# Autodesk Inventor assembly: Full Chassis with Arduino, Gyro, 1 inch Arms, and Konylak Wheels
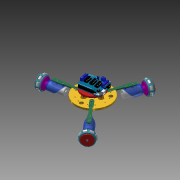
[picture p0: Inventor's stored thumbnail of the model, 180x180]
Saved by Autodesk Inventor 2014 (Build 180170000, 170)
## iProperties
Created: 2014-02-14
Part Number: Full Chassis with Arduino, Gyro, 1 inch Arms, and Konylak Wheels
Document SubType Name: Assembly
Designer: Spooner
Author: Spooner
## Documents named in this file (6)
- C:\Users\Spooner\Documents\Inventor\FerretBall Robot\3Pod\Inventor 2014 Files\Full Chassis with Arduino, Gyro, 1 inch Arms, and Konylak Wheels.iam
- C:\Users\Spooner\Documents\Inventor\FerretBall Robot\3Pod\Inventor 2014 Files\Main Body with Arduino and Gyro Mounts.iam
- C:\Users\Spooner\Documents\Inventor\Content Center Files\R2014\en-US\JIS B 1111(1)\JIS B 1111 - M3x10(1).ipt
- C:\Users\Spooner\Documents\Inventor\Content Center Files\R2014\en-US\JIS B 1181 U\JIS B 1181 - B M3.ipt
- C:\Users\Spooner\Documents\Inventor\FerretBall Robot\3Pod\Inventor 2014 Files\Full Motor Arm (1 inch) with Kornylak Wheel.iam
- C:\Users\Spooner\Documents\Inventor\FerretBall Robot\3Pod\Inventor 2014 Files\Adafruit Motor Sheild 1.2.ipt
## Components (17 placed, 5 different names)
1. Main Body with Arduino and Gyro Mounts:1 [sub-assembly] — Insert:10, Insert:11, Insert:12, Insert:13, Insert:14, Insert:15, Insert:16, Insert:17, Insert:18, Mate:4, Angle:7, Mate:5
2. JIS B 1111 M3x10:1 — Insert:11, Mate:3
3. JIS B 1111 M3x10:2 — Insert:10
4. JIS B 1111 M3x10:3 — Insert:15, Mate:1
5. JIS B 1111 M3x10:4 — Insert:14
6. JIS B 1111 M3x10:5 — Insert:13, Mate:2
7. JIS B 1111 M3x10:6 — Insert:12
8. JIS B 1181 (unchamfered) - Metric B M3:1 — Insert:21, Angle:1
9. JIS B 1181 (unchamfered) - Metric B M3:2 — Insert:24, Angle:6
10. JIS B 1181 (unchamfered) - Metric B M3:3 — Insert:19, Angle:2
11. JIS B 1181 (unchamfered) - Metric B M3:4 — Insert:20, Angle:3
12. JIS B 1181 (unchamfered) - Metric B M3:5 — Insert:22, Angle:4
13. JIS B 1181 (unchamfered) - Metric B M3:6 — Insert:23, Angle:5
14. Full Motor Arm (1 inch) with Kornylak Wheel:1 [sub-assembly] — Insert:18, Mate:3, Insert:21, Angle:1, Insert:24, Angle:6
15. Full Motor Arm (1 inch) with Kornylak Wheel:2 [sub-assembly] — Insert:17, Mate:2, Insert:22, Insert:23, Angle:4, Angle:5
16. Full Motor Arm (1 inch) with Kornylak Wheel:3 [sub-assembly] — Insert:16, Mate:1, Insert:19, Insert:20, Angle:2, Angle:3
17. Adafruit Motor Sheild 1.2:1 — Mate:4, Angle:7, Mate:5
## Relationships (27: Insert 15, Angle 7, Mate 5)
- Insert:10: Main Body with Arduino and Gyro Mounts:1 ↔ JIS B 1111 M3x10:2
- Insert:11: Main Body with Arduino and Gyro Mounts:1 ↔ JIS B 1111 M3x10:1
- Insert:12: Main Body with Arduino and Gyro Mounts:1 ↔ JIS B 1111 M3x10:6
- Insert:13: Main Body with Arduino and Gyro Mounts:1 ↔ JIS B 1111 M3x10:5
- Insert:14: Main Body with Arduino and Gyro Mounts:1 ↔ JIS B 1111 M3x10:4
- Insert:15: Main Body with Arduino and Gyro Mounts:1 ↔ JIS B 1111 M3x10:3
- Insert:16: Main Body with Arduino and Gyro Mounts:1 ↔ Full Motor Arm (1 inch) with Kornylak Wheel:3
- Mate:1: JIS B 1111 M3x10:3 ↔ Full Motor Arm (1 inch) with Kornylak Wheel:3
- Insert:17: Main Body with Arduino and Gyro Mounts:1 ↔ Full Motor Arm (1 inch) with Kornylak Wheel:2
- Mate:2: JIS B 1111 M3x10:5 ↔ Full Motor Arm (1 inch) with Kornylak Wheel:2
- Insert:18: Main Body with Arduino and Gyro Mounts:1 ↔ Full Motor Arm (1 inch) with Kornylak Wheel:1
- Mate:3: JIS B 1111 M3x10:1 ↔ Full Motor Arm (1 inch) with Kornylak Wheel:1
- Insert:19: JIS B 1181 (unchamfered) - Metric B M3:3 ↔ Full Motor Arm (1 inch) with Kornylak Wheel:3
- Insert:20: JIS B 1181 (unchamfered) - Metric B M3:4 ↔ Full Motor Arm (1 inch) with Kornylak Wheel:3
- Insert:21: JIS B 1181 (unchamfered) - Metric B M3:1 ↔ Full Motor Arm (1 inch) with Kornylak Wheel:1
- Insert:22: JIS B 1181 (unchamfered) - Metric B M3:5 ↔ Full Motor Arm (1 inch) with Kornylak Wheel:2
- Insert:23: JIS B 1181 (unchamfered) - Metric B M3:6 ↔ Full Motor Arm (1 inch) with Kornylak Wheel:2
- Angle:1 (0 deg): JIS B 1181 (unchamfered) - Metric B M3:1 ↔ Full Motor Arm (1 inch) with Kornylak Wheel:1
- Angle:2 (0 deg): JIS B 1181 (unchamfered) - Metric B M3:3 ↔ Full Motor Arm (1 inch) with Kornylak Wheel:3
- Angle:3 (0 deg): JIS B 1181 (unchamfered) - Metric B M3:4 ↔ Full Motor Arm (1 inch) with Kornylak Wheel:3
- Angle:4 (0 deg): JIS B 1181 (unchamfered) - Metric B M3:5 ↔ Full Motor Arm (1 inch) with Kornylak Wheel:2
- Angle:5 (0 deg): JIS B 1181 (unchamfered) - Metric B M3:6 ↔ Full Motor Arm (1 inch) with Kornylak Wheel:2
- Insert:24: JIS B 1181 (unchamfered) - Metric B M3:2 ↔ Full Motor Arm (1 inch) with Kornylak Wheel:1
- Angle:6 (0 deg): JIS B 1181 (unchamfered) - Metric B M3:2 ↔ Full Motor Arm (1 inch) with Kornylak Wheel:1
- Mate:4: Main Body with Arduino and Gyro Mounts:1 ↔ Adafruit Motor Sheild 1.2:1
- Angle:7 (0 deg): Main Body with Arduino and Gyro Mounts:1 ↔ Adafruit Motor Sheild 1.2:1
- Mate:5: Main Body with Arduino and Gyro Mounts:1 ↔ Adafruit Motor Sheild 1.2:1
